# Autodesk Inventor assembly: nhk36
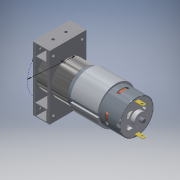
[picture p0: Inventor's stored thumbnail of the model, 180x180]
Saved by Autodesk Inventor 2019 (Build 230136000, 136)
## iProperties
Created: 2022-02-27
Part Number: nhk36
Material: 一般
Document SubType Name: Assembly
Designer: yuta
Author: yuta
## Documents named in this file (5)
- C:\Users\yuta\Documents\NHK\nhk36.iam
- C:\Users\yuta\Documents\NHK\nhk28.ipt
- C:\Users\yuta\Documents\NHK\nhk29.ipt
- C:\Users\yuta\Documents\NHK\RS775+gennsoku.iam
- C:\Users\yuta\Documents\NHK\nhk30.ipt
## Components (5 placed, 4 different names)
1. nhk28:1 — メイト:1, フラッシュ:1, フラッシュ:2, メイト:2, フラッシュ:3, フラッシュ:4, メイト:3, フラッシュ:5
2. nhk29:1 — メイト:2, フラッシュ:3, フラッシュ:4
3. nhk29:2 — メイト:1, フラッシュ:1, フラッシュ:2, メイト:4, メイト:6
4. RS775+gennsoku:1 [sub-assembly] — メイト:3, フラッシュ:5
5. nhk30:1 — メイト:4, メイト:6
## Relationships (10: Mate 5, Flush 5)
- メイト:1 [Mate]: nhk28:1 ↔ nhk29:2
- フラッシュ:1 [Flush]: nhk28:1 ↔ nhk29:2
- フラッシュ:2 [Flush]: nhk28:1 ↔ nhk29:2
- メイト:2 [Mate]: nhk28:1 ↔ nhk29:1
- フラッシュ:3 [Flush]: nhk28:1 ↔ nhk29:1
- フラッシュ:4 [Flush]: nhk28:1 ↔ nhk29:1
- メイト:3 [Mate]: nhk28:1 ↔ RS775+gennsoku:1
- フラッシュ:5 [Flush]: nhk28:1 ↔ RS775+gennsoku:1
- メイト:4 [Mate]: nhk29:2 ↔ nhk30:1
- メイト:6 [Mate]: nhk29:2 ↔ nhk30:1
